# Autodesk Inventor assembly: 17-0028-0099
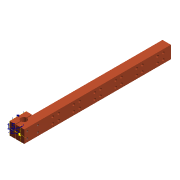
[picture p0: Inventor's stored thumbnail of the model, 180x180]
Saved by Autodesk Inventor 2016 SP2 (Build 200236200, 236)
## iProperties
Category: -
Company: Universiteit van Amsterdam
Created: 2017-12-07
Part Number: 17-0028-0099
Document SubType Name: Assembly
Designer: Daan Giesen
Project: Digital PID Loop
Cost Center: 17-0028
User Status: Work in Progress
Authority: Reichsöllner, Lukas
Author: Daan Giesen
Title: Digital PID Loop
Revision Number: A
## Documents named in this file (4)
- D:\VaultLocalWorkingFolder\UvA_MT\Projects\2017\17-0028 Digital PID Loop\10_Assemblies\17-0028-0099.iam
- D:\VaultLocalWorkingFolder\UvA_MT\Projects\2017\17-0028 Digital PID Loop\20_3D-Models\17-0028-0100.ipt
- D:\VaultLocalWorkingFolder\UvA_MT\Projects\2017\17-0028 Digital PID Loop\20_3D-Models\17-0028-0101.ipt
- D:\VaultLocalWorkingFolder\UvA_MT\Projects\2017\17-0028 Digital PID Loop\10_Assemblies\17-0028-0099\Design Accelerator\17-0028-0107.iam
## Components (3 placed, 3 different names)
1. 17-0028-0100:1 — Mate:1, Mate:2
2. 17-0028-0101:1
3. Bolted Connection:1 [sub-assembly] — Mate:1, Mate:2
## Relationships (2: Mate 2)
- Mate:1: 17-0028-0100:1 ↔ Bolted Connection:1
- Mate:2: 17-0028-0100:1 ↔ Bolted Connection:1
